# Autodesk Inventor assembly: sistema embebido
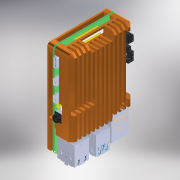
[picture p0: Inventor's stored thumbnail of the model, 180x180]
Saved by Autodesk Inventor 2021.4 (Build 254397000, 397)
## iProperties
Created: 2022-12-03
Part Number: sistema embebido
Document SubType Name: Assembly
Designer: user
Author: user
## Documents named in this file (5)
- C:\Users\crist\OneDrive - Escuela Superior Politécnica del Litoral\Escritorio\Archivos\Dron\Raspberry Pi\sistema embebido final.iam
- C:\Users\crist\OneDrive - Escuela Superior Politécnica del Litoral\Escritorio\Archivos\Dron\Raspberry Pi\Assembly Raspberry Pi 4 B.iam
- C:\Users\crist\OneDrive - Escuela Superior Politécnica del Litoral\Escritorio\Archivos\Dron\Raspberry Pi\Heat sink.ipt
- C:\Users\crist\OneDrive - Escuela Superior Politécnica del Litoral\Escritorio\Archivos\Dron\Raspberry Pi\Heatsink Base.ipt
- C:\Users\crist\OneDrive - Escuela Superior Politécnica del Litoral\Escritorio\Archivos\Dron\Raspberry Pi\jumper.ipt
## Components (13 placed, 4 different names)
1. Assembly Raspberry Pi 4 B:1 [sub-assembly] — Coincidencia:1, Coincidencia:2, Nivelación:1, Nivelación:2, Nivelación:3, Nivelación:4, Coincidencia:17, Coincidencia:18, Coincidencia:19, Coincidencia:20, Coincidencia:21, Coincidencia:22, Coincidencia:23, Coincidencia:24, Coincidencia:25, Coincidencia:26, Coincidencia:27, Coincidencia:28, Coincidencia:29, Coincidencia:30, Coincidencia:31, Coincidencia:32, Coincidencia:33, Coincidencia:34, Coincidencia:35, Coincidencia:36
2. Heat sink:1 — Coincidencia:2, Nivelación:1, Nivelación:4
3. Heatsink Base:1 — Coincidencia:1, Nivelación:2, Nivelación:3
4. jumper:4 — Coincidencia:23, Coincidencia:24
5. jumper:5 — Coincidencia:25, Coincidencia:26
6. jumper:6 — Coincidencia:27, Coincidencia:28
7. jumper:7 — Coincidencia:19, Coincidencia:20
8. jumper:9 — Coincidencia:21, Coincidencia:22
9. jumper:10 — Coincidencia:17, Coincidencia:18
10. jumper:11 — Coincidencia:31, Coincidencia:32
11. jumper:12 — Coincidencia:33, Coincidencia:34
12. jumper:13 — Coincidencia:35, Coincidencia:36
13. jumper:14 — Coincidencia:29, Coincidencia:30
## Relationships (28: Mate 24, Flush 4)
- Coincidencia:1 [Mate]: Assembly Raspberry Pi 4 B:1 ↔ Heatsink Base:1
- Coincidencia:2 [Mate]: Assembly Raspberry Pi 4 B:1 ↔ Heat sink:1
- Nivelación:1 [Flush]: Assembly Raspberry Pi 4 B:1 ↔ Heat sink:1
- Nivelación:2 [Flush]: Assembly Raspberry Pi 4 B:1 ↔ Heatsink Base:1
- Nivelación:3 [Flush]: Assembly Raspberry Pi 4 B:1 ↔ Heatsink Base:1
- Nivelación:4 [Flush]: Assembly Raspberry Pi 4 B:1 ↔ Heat sink:1
- Coincidencia:8 [Mate]
- Coincidencia:9 [Mate]
- Coincidencia:17 [Mate]: Assembly Raspberry Pi 4 B:1 ↔ jumper:10
- Coincidencia:18 [Mate]: Assembly Raspberry Pi 4 B:1 ↔ jumper:10
- Coincidencia:19 [Mate]: Assembly Raspberry Pi 4 B:1 ↔ jumper:7
- Coincidencia:20 [Mate]: Assembly Raspberry Pi 4 B:1 ↔ jumper:7
- Coincidencia:21 [Mate]: Assembly Raspberry Pi 4 B:1 ↔ jumper:9
- Coincidencia:22 [Mate]: Assembly Raspberry Pi 4 B:1 ↔ jumper:9
- Coincidencia:23 [Mate]: Assembly Raspberry Pi 4 B:1 ↔ jumper:4
- Coincidencia:24 [Mate]: Assembly Raspberry Pi 4 B:1 ↔ jumper:4
- Coincidencia:25 [Mate]: Assembly Raspberry Pi 4 B:1 ↔ jumper:5
- Coincidencia:26 [Mate]: Assembly Raspberry Pi 4 B:1 ↔ jumper:5
- Coincidencia:27 [Mate]: Assembly Raspberry Pi 4 B:1 ↔ jumper:6
- Coincidencia:28 [Mate]: Assembly Raspberry Pi 4 B:1 ↔ jumper:6
- Coincidencia:29 [Mate]: Assembly Raspberry Pi 4 B:1 ↔ jumper:14
- Coincidencia:30 [Mate]: Assembly Raspberry Pi 4 B:1 ↔ jumper:14
- Coincidencia:31 [Mate]: Assembly Raspberry Pi 4 B:1 ↔ jumper:11
- Coincidencia:32 [Mate]: Assembly Raspberry Pi 4 B:1 ↔ jumper:11
- Coincidencia:33 [Mate]: Assembly Raspberry Pi 4 B:1 ↔ jumper:12
- Coincidencia:34 [Mate]: Assembly Raspberry Pi 4 B:1 ↔ jumper:12
- Coincidencia:35 [Mate]: Assembly Raspberry Pi 4 B:1 ↔ jumper:13
- Coincidencia:36 [Mate]: Assembly Raspberry Pi 4 B:1 ↔ jumper:13
